# Autodesk Inventor assembly: AMD Ryzen CPU
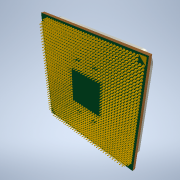
[picture p0: Inventor's stored thumbnail of the model, 180x180]
Saved by Autodesk Inventor 2020 (Build 240168000, 168)
## iProperties
Created: 2020-11-28
Part Number: AMD Ryzen CPU
Document SubType Name: Assembly
Designer: david
Author: david
## Documents named in this file (3)
- \\192.168.178.2\David\Documents\Inventor\zeichnungen\Mini mini ITX PC\Ryzen\AMD Ryzen CPU.iam
- \\192.168.178.2\David\Documents\Inventor\zeichnungen\Mini mini ITX PC\Ryzen\Ryzen PCB.ipt
- \\192.168.178.2\David\Documents\Inventor\zeichnungen\Mini mini ITX PC\Ryzen\Ryzen IHS.ipt
## Components (2 placed, 2 different names)
1. Ryzen PCB:1 — Passend:1, Passend:2, Passend:3
2. Ryzen IHS:1 — Passend:1, Passend:2, Passend:3
## Relationships (3: Mate 3)
- Passend:1 [Mate]: Ryzen PCB:1 ↔ Ryzen IHS:1
- Passend:2 [Mate]: Ryzen PCB:1 ↔ Ryzen IHS:1
- Passend:3 [Mate]: Ryzen PCB:1 ↔ Ryzen IHS:1
